# Autodesk Inventor assembly: Assembled box
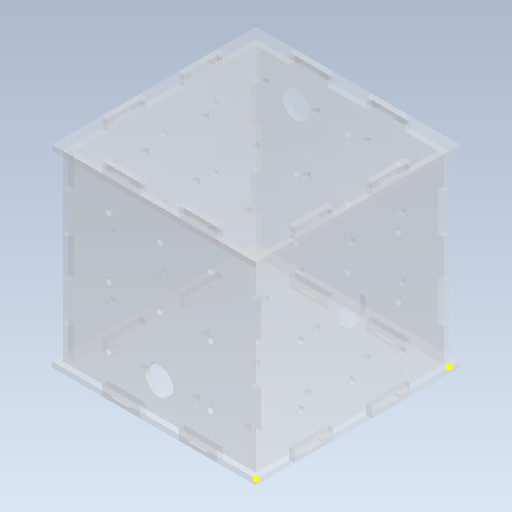
[picture p0: Inventor's stored thumbnail of the model, 512x512]
Saved by Autodesk Inventor 2020 (Build 240168000, 168)
## iProperties
Created: 2020-02-27
Part Number: Assembled box
Document SubType Name: Assembly
Designer: jstr255
Author: jstr255
## Documents named in this file (7)
- C:\Users\jstr255\Documents\Inventor\Project A\Group boxes\Group 14\Assembled box.iam
- C:\Users\jstr255\Documents\Inventor\Project A\Group boxes\Group 14\Box base.ipt
- C:\Users\jstr255\Documents\Inventor\Project A\Group boxes\Group 14\Box side 1.ipt
- C:\Users\jstr255\Documents\Inventor\Project A\Group boxes\Group 14\Box side 2.ipt
- C:\Users\jstr255\Documents\Inventor\Project A\Group boxes\Group 14\Box side 3.ipt
- C:\Users\jstr255\Documents\Inventor\Project A\Group boxes\Group 14\Box side 4.ipt
- C:\Users\jstr255\Documents\Inventor\Project A\Group boxes\Group 14\Box top.ipt
## Components (6 placed, 6 different names)
1. Box base:1 — Mate:1, Mate:2, Mate:3, Mate:4, Mate:5, Mate:6, Mate:7, Mate:8, Mate:9, Mate:10
2. Box side 1:1 — Mate:1, Mate:2, Mate:3, Flush:1, Mate:14
3. Box side 2:1 — Mate:4, Mate:5, Mate:6, Mate:13
4. Box side 3:1 — Mate:7, Mate:8, Mate:9, Mate:11
5. Box side 4:1 — Mate:10, Mate:11, Flush:1, Mate:12
6. Box top:1 — Mate:12, Mate:13, Mate:14
## Relationships (15: Mate 14, Flush 1)
- Mate:1: Box base:1 ↔ Box side 1:1
- Mate:2: Box base:1 ↔ Box side 1:1
- Mate:3: Box base:1 ↔ Box side 1:1
- Mate:4: Box base:1 ↔ Box side 2:1
- Mate:5: Box base:1 ↔ Box side 2:1
- Mate:6: Box base:1 ↔ Box side 2:1
- Mate:7: Box base:1 ↔ Box side 3:1
- Mate:8: Box base:1 ↔ Box side 3:1
- Mate:9: Box base:1 ↔ Box side 3:1
- Mate:10: Box base:1 ↔ Box side 4:1
- Mate:11: Box side 3:1 ↔ Box side 4:1
- Flush:1: Box side 1:1 ↔ Box side 4:1
- Mate:12: Box side 4:1 ↔ Box top:1
- Mate:13: Box side 2:1 ↔ Box top:1
- Mate:14: Box side 1:1 ↔ Box top:1
